# Autodesk Inventor assembly: VacuumTubeHolder
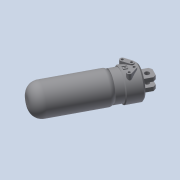
[picture p0: Inventor's stored thumbnail of the model, 180x180]
Saved by Autodesk Inventor 2020 (Build 240168000, 168)
## iProperties
Created: 2015-06-28
Part Number: VacuumTubeHolder
Document SubType Name: Assembly
Designer: Val
Author: Val
## Documents named in this file (3)
- C:\Users\Val\Desktop\drummingrobot\src\parts\VacuumTubeHolder.iam
- C:\Users\Val\Desktop\drummingrobot\src\parts\VacuumTubeHolderBase.ipt
- C:\Users\Val\Desktop\drummingrobot\src\parts\external\VacuumTube6L6GCSTR440.ipt
## Components (2 placed, 2 different names)
1. VacuumTubeHolderBase:1 — Mate:3, Mate:4
2. VacuumTube:1 — Mate:3, Mate:4
## Relationships (2: Mate 2)
- Mate:3 (-6.5 mm): VacuumTubeHolderBase:1 ↔ VacuumTube:1
- Mate:4: VacuumTubeHolderBase:1 ↔ VacuumTube:1
